# Autodesk Inventor assembly: Batteriepack
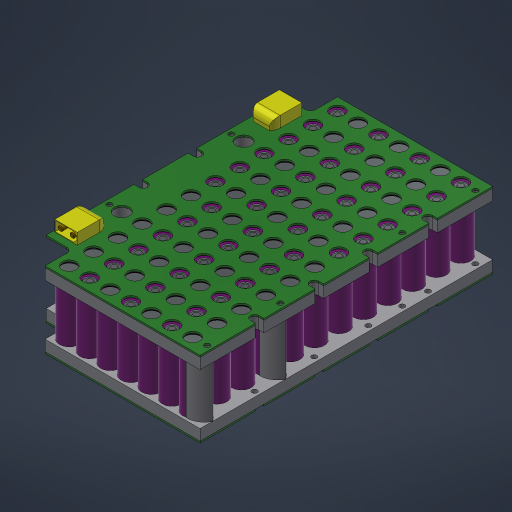
[picture p0: Inventor's stored thumbnail of the model, 512x512]
Saved by Autodesk Inventor 2023.5 (Build 275446000, 446)
## iProperties
Created: 2025-03-26
Part Number: Batteriepack
Document SubType Name: Assembly
Designer: David Lill
Author: David Lill
## Documents named in this file (8)
- C:\Users\David\Documents\Inventor\E-16 Batterie\Batteriepack.iam
- C:\Users\David\Documents\Inventor\E-16 Batterie\Platte1.ipt
- C:\Users\David\Documents\Inventor\E-16 Batterie\PCB.ipt
- C:\Users\David\Documents\Inventor\E-16 Batterie\18650.ipt
- C:\Users\David\Documents\Inventor\E-16 Batterie\Platte2.ipt
- C:\Users\David\Documents\Inventor\E-16 Batterie\XT90PW.ipt
- C:\Users\David\Documents\Inventor\E-16 Batterie\Abstandhalter.ipt
- C:\Users\David\Documents\Inventor\E-16 Batterie\Abstandhalter_2.ipt
## Components (94 placed, 7 different names)
1. Platte1:3 — Einfügen:1, Einfügen:2, Einfügen:5, Einfügen:6, Einfügen:7, Einfügen:8, Einfügen:17, Einfügen:18, Einfügen:19, Einfügen:20, Einfügen:21, Einfügen:22
2. PCB:1 — Einfügen:1, Einfügen:2
3. PCB:2 — Einfügen:11, Einfügen:12, Einfügen:13, Einfügen:14, Einfügen:15, Einfügen:16
4. Platte2:1 — Einfügen:9, Einfügen:10, Einfügen:11, Einfügen:12
5. XT90PW:1 — Einfügen:15, Einfügen:16
6. XT90PW:2 — Einfügen:13, Einfügen:14
7. Abstandhalter:1 — Einfügen:17, Einfügen:18
8. Abstandhalter:2 — Einfügen:19, Einfügen:20
9. Abstandhalter_2:1 — Passend:1, Einfügen:21
10. Abstandhalter_2:2 — Passend:2, Einfügen:22
11. 18650:1 — Einfügen:5, Einfügen:10
12. 18650:4 — Einfügen:8
13. 18650:5
14. 18650:6
15. 18650:7
16. 18650:8
17. 18650:9
18. 18650:10
19. 18650:11
20. 18650:12
21. 18650:13
22. 18650:14
23. 18650:25
24. 18650:26
25. 18650:27
26. 18650:28
27. 18650:29
28. 18650:30
29. 18650:31
30. 18650:32
31. 18650:33
32. 18650:34
33. 18650:35
34. 18650:36
35. 18650:37
36. 18650:38
37. 18650:39
38. 18650:40
39. 18650:41
40. 18650:42
41. 18650:43
42. 18650:44
43. 18650:45
44. 18650:46
45. 18650:47
46. 18650:48
47. 18650:49 — Passend:1
48. 18650:50
49. 18650:51
50. 18650:52
51. 18650:53
52. 18650:54
53. 18650:55 — Passend:2
54. 18650:56
55. 18650:57
56. 18650:58
57. 18650:59
58. 18650:60 — Einfügen:9
59. 18650:2 — Einfügen:7
60. 18650:3 — Einfügen:6
61. 18650:15
62. 18650:16
63. 18650:17
64. 18650:18
65. 18650:19
66. 18650:20
67. 18650:21
68. 18650:22
69. 18650:23
70. 18650:24
71. 18650:61
72. 18650:62
73. 18650:63
74. 18650:64
75. 18650:65
76. 18650:66
77. 18650:67
78. 18650:68
79. 18650:69
80. 18650:70
81. 18650:71
82. 18650:72
83. 18650:73
84. 18650:74
85. 18650:75
86. 18650:76
87. 18650:77
88. 18650:78
89. 18650:79
90. 18650:80
91. 18650:81
92. 18650:82
93. 18650:83
94. 18650:84
## Component patterns: (4 elements), (3 elements), (6 elements, first: 18650:1 + 18650:4), Komponentenanordnung 5:2 (6 elements), Komponentenanordnung 5:3 (6 elements), Komponentenanordnung 5:4 (6 elements), (6 elements, first: 18650:2 + 18650:3), Komponentenanordnung 6:2 (6 elements), Komponentenanordnung 6:3 (6 elements)
## Relationships (22: Insert 20, Mate 2)
- Einfügen:1 [Insert]: Platte1:3 ↔ PCB:1
- Einfügen:2 [Insert]: Platte1:3 ↔ PCB:1
- Einfügen:5 [Insert]: Platte1:3 ↔ 18650:1
- Einfügen:6 [Insert]: Platte1:3 ↔ 18650:3
- Einfügen:7 [Insert]: Platte1:3 ↔ 18650:2
- Einfügen:8 [Insert]: Platte1:3 ↔ 18650:4
- Einfügen:9 [Insert]: Platte2:1 ↔ 18650:60
- Einfügen:10 [Insert]: Platte2:1 ↔ 18650:1
- Einfügen:11 [Insert]: PCB:2 ↔ Platte2:1
- Einfügen:12 [Insert]: PCB:2 ↔ Platte2:1
- Einfügen:13 [Insert]: PCB:2 ↔ XT90PW:2
- Einfügen:14 [Insert]: PCB:2 ↔ XT90PW:2
- Einfügen:15 [Insert]: PCB:2 ↔ XT90PW:1
- Einfügen:16 [Insert]: PCB:2 ↔ XT90PW:1
- Einfügen:17 [Insert]: Platte1:3 ↔ Abstandhalter:1
- Einfügen:18 [Insert]: Platte1:3 ↔ Abstandhalter:1
- Einfügen:19 [Insert]: Platte1:3 ↔ Abstandhalter:2
- Einfügen:20 [Insert]: Platte1:3 ↔ Abstandhalter:2
- Passend:1 [Mate]: Abstandhalter_2:1 ↔ 18650:49
- Passend:2 [Mate]: Abstandhalter_2:2 ↔ 18650:55
- Einfügen:21 [Insert]: Platte1:3 ↔ Abstandhalter_2:1
- Einfügen:22 [Insert]: Platte1:3 ↔ Abstandhalter_2:2
